# Autodesk Inventor assembly: Shapeoko_v2.0_500
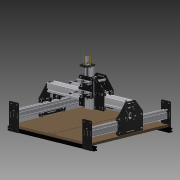
[picture p0: Inventor's stored thumbnail of the model, 180x180]
Saved by Autodesk Inventor 2014 (Build 180170000, 170)
## iProperties
Created: 2013-09-18
Part Number: Shapeoko_v2.0_500
Document SubType Name: Assembly
Designer: Edward
Author: Edward
## Documents named in this file (7)
- C:\Users\Edward\Documents\GitHub\Shapeoko_2\Shapeoko_2.iam
- C:\Users\Edward\Documents\GitHub\Shapeoko_2\25287-02.ipt
- C:\Users\Edward\Documents\GitHub\Shapeoko_2\25286-01.ipt
- C:\Users\Edward\Documents\GitHub\Shapeoko_2\26016-01.ipt
- C:\Users\Edward\Documents\GitHub\Shapeoko_2\S2_Yaxis_Rail_500.iam
- C:\Users\Edward\Documents\GitHub\Shapeoko_2\S2_Xaxis_500.iam
- C:\Users\Edward\Documents\GitHub\Shapeoko_2\S2_Work_Area_500.iam
## Components (28 placed, 6 different names)
1. S2_Work_Area_500:1 [sub-assembly] — Mate:1, Flush:1, Mate:2, Flush:2, Flush:4
2. S2_Yaxis_Rail_500:1 [sub-assembly] — Mate:2, Flush:2, Mate:4, Flush:3, Insert:3, Insert:6, Flush:4
3. S2_Yaxis_Rail_500:2 [sub-assembly] — Mate:1, Flush:1, Mate:3
4. S2_Xaxis_500:1 [sub-assembly] — Mate:3, Mate:4, Flush:3
5. 26016-01:1
6. 25287-02:1 — Insert:3
7. 25286-01:1
8. 26016-01:2
9. 25287-02:2
10. 25286-01:2
11. 26016-01:3
12. 25287-02:3
13. 25286-01:3
14. 26016-01:4
15. 25287-02:4
16. 25286-01:4
17. 25287-02:5 — Insert:6
18. 25286-01:5
19. 26016-01:5
20. 25287-02:6
21. 25286-01:6
22. 26016-01:6
23. 25287-02:7
24. 25286-01:7
25. 26016-01:7
26. 25287-02:8
27. 25286-01:8
28. 26016-01:8
## Component patterns: Front_fasteners (2 elements), Rear Fasteners (2 elements), (2 elements, first: 26016-01:1 + 25287-02:1 + 25286-01:1), Component Pattern 1:2 (2 elements), (2 elements, first: 25287-02:5 + 25286-01:5 + 26016-01:5), Component Pattern 3:2 (2 elements)
## Relationships (14: Insert 6, Mate 4, Flush 4)
- Mate:1: S2_Work_Area_500:1 ↔ S2_Yaxis_Rail_500:2
- Flush:1: S2_Work_Area_500:1 ↔ S2_Yaxis_Rail_500:2
- Mate:2: S2_Work_Area_500:1 ↔ S2_Yaxis_Rail_500:1
- Flush:2: S2_Work_Area_500:1 ↔ S2_Yaxis_Rail_500:1
- Mate:3 (6.35 mm): S2_Yaxis_Rail_500:2 ↔ S2_Xaxis_500:1
- Mate:4 (6.35 mm): S2_Yaxis_Rail_500:1 ↔ S2_Xaxis_500:1
- Flush:3 (-25 mm): S2_Yaxis_Rail_500:1 ↔ S2_Xaxis_500:1
- [Insert]: 25287-02:1 ↔ 25286-01:1
- [Insert] (5.416 mm): 26016-01:1 ↔ 25287-02:1
- Insert:3: S2_Yaxis_Rail_500:1 ↔ 25287-02:1
- [Insert]: 25287-02:5 ↔ 25286-01:5
- [Insert] (5.416 mm): 25287-02:5 ↔ 26016-01:5
- Insert:6: S2_Yaxis_Rail_500:1 ↔ 25287-02:5
- Flush:4 (11.35 mm): S2_Work_Area_500:1 ↔ S2_Yaxis_Rail_500:1
## Named parameters: d128_d120 = 0 mm, d129_d123 = 5.416 mm, d22_d128_d120 = 0 mm, d23_d129_d123 = 5.416 mm
